# Autodesk Inventor assembly: PK_Arm_V2
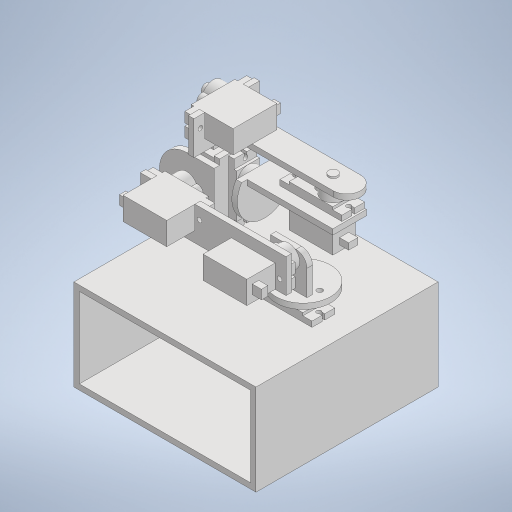
[picture p0: Inventor's stored thumbnail of the model, 512x512]
Saved by Autodesk Inventor 2023 (Build 270158000, 158)
## iProperties
Created: 2022-04-08
Part Number: PK_Arm_V2
Document SubType Name: Assembly
Designer: device
Author: device
## Documents named in this file (9)
- D:\NTNU\PK_Arm_V2\PK_Arm_V2.iam
- D:\NTNU\PK_Arm_V2\base_box.ipt
- D:\NTNU\PK_Arm_V2\MG90.ipt
- D:\NTNU\PK_Arm_V2\Pad_1.ipt
- D:\NTNU\PK_Arm_V2\Arm_1.ipt
- D:\NTNU\PK_Arm_V2\Pad_2.ipt
- D:\NTNU\PK_Arm_V2\Arm_2.ipt
- D:\NTNU\PK_Arm_V2\Arm_3.ipt
- D:\NTNU\PK_Arm_V2\Eazy-Card.ipt
## Components (13 placed, 8 different names)
1. Eazy-Card:1
2. base_box:1 — 貼合:26, 貼合:27, 貼合:28
3. MG90:1 — 貼合:1, 貼合:2, 貼合:26, 貼合:27, 貼合:28, 角度:1
4. MG90:2 — 貼合:3, 貼合:4, 角度:2, 貼合:5, 貼合:6, 貼合:7
5. Pad_1:1 — 貼合:1, 貼合:2, 貼合:3, 貼合:4, 角度:1, 角度:2
6. Arm_1:1 — 貼合:5, 貼合:6, 貼合:7, 貼合:8, 貼合:9, 貼合:10, 角度:3
7. MG90:3 — 貼合:8, 貼合:9, 貼合:10, 貼合:11, 貼合:12
8. Pad_2:1 — 貼合:11, 貼合:12, 貼合:13, 貼合:14, 貼合:15, 角度:3
9. MG90:4 — 貼合:13, 貼合:14, 貼合:15, 貼合:19, 貼合:20, 角度:4
10. Arm_2:1 — 貼合:16, 貼合:17, 貼合:18, 貼合:19, 貼合:20, 角度:4
11. MG90:5 — 貼合:16, 貼合:17, 貼合:18, 貼合:21, 貼合:22, 角度:5
12. Arm_3:1 — 貼合:21, 貼合:22, 角度:5, 貼合:23, 貼合:24, 貼合:25
13. MG90:6 — 貼合:23, 貼合:24, 貼合:25
## Relationships (33: Mate 28, Angle 5)
- 貼合:1 [Mate]: MG90:1 ↔ Pad_1:1
- 貼合:2 [Mate]: MG90:1 ↔ Pad_1:1
- 貼合:3 [Mate]: MG90:2 ↔ Pad_1:1
- 貼合:4 [Mate]: MG90:2 ↔ Pad_1:1
- 貼合:5 [Mate]: MG90:2 ↔ Arm_1:1
- 貼合:6 [Mate]: MG90:2 ↔ Arm_1:1
- 貼合:7 [Mate]: MG90:2 ↔ Arm_1:1
- 貼合:8 [Mate]: Arm_1:1 ↔ MG90:3
- 貼合:9 [Mate]: Arm_1:1 ↔ MG90:3
- 貼合:10 [Mate]: Arm_1:1 ↔ MG90:3
- 貼合:11 [Mate]: MG90:3 ↔ Pad_2:1
- 貼合:12 [Mate]: MG90:3 ↔ Pad_2:1
- 貼合:13 [Mate]: Pad_2:1 ↔ MG90:4
- 貼合:14 [Mate]: Pad_2:1 ↔ MG90:4
- 貼合:15 [Mate]: Pad_2:1 ↔ MG90:4
- 貼合:16 [Mate]: Arm_2:1 ↔ MG90:5
- 貼合:17 [Mate]: Arm_2:1 ↔ MG90:5
- 貼合:18 [Mate]: Arm_2:1 ↔ MG90:5
- 貼合:19 [Mate]: MG90:4 ↔ Arm_2:1
- 貼合:20 [Mate]: MG90:4 ↔ Arm_2:1
- 貼合:21 [Mate]: MG90:5 ↔ Arm_3:1
- 貼合:22 [Mate]: MG90:5 ↔ Arm_3:1
- 貼合:23 [Mate]: Arm_3:1 ↔ MG90:6
- 貼合:24 [Mate]: Arm_3:1 ↔ MG90:6
- 貼合:26 [Mate]: base_box:1 ↔ MG90:1
- 貼合:25 [Mate]: Arm_3:1 ↔ MG90:6
- 貼合:27 [Mate]: base_box:1 ↔ MG90:1
- 貼合:28 [Mate]: base_box:1 ↔ MG90:1
- 角度:1 [Angle] (0 deg): MG90:1 ↔ Pad_1:1
- 角度:2 [Angle] (0 deg): MG90:2 ↔ Pad_1:1
- 角度:3 [Angle] (0 deg): Arm_1:1 ↔ Pad_2:1
- 角度:4 [Angle] (0 deg): MG90:4 ↔ Arm_2:1
- 角度:5 [Angle] (0 deg): MG90:5 ↔ Arm_3:1
## Named parameters: w = 3 mm
